# Autodesk Inventor assembly: センサ2セット積み左
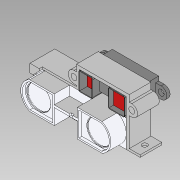
[picture p0: Inventor's stored thumbnail of the model, 180x180]
Saved by Autodesk Inventor 2017 (Build 210142000, 142)
## iProperties
Part Number: センサ2セット積み左
Material: 一般
Document SubType Name: Assembly
Designer: HISAAKI
Author: HISAAKI
## Documents named in this file (4)
- C:\Users\HISAAKI\Documents\LYNCS\CanSat\2017種子島\cansat-structure\センサ2セット積み左.iam
- C:\Users\HISAAKI\Documents\LYNCS\CanSat\2017種子島\cansat-structure\Sharp_2Y0A710.ipt
- C:\Users\HISAAKI\Documents\LYNCS\CanSat\2017種子島\cansat-structure\SharpDistanceRanger.ipt
- C:\Users\HISAAKI\Documents\LYNCS\CanSat\2017種子島\cansat-structure\センサ冶具.ipt
## Components (3 placed, 3 different names)
1. センサ冶具:1 — メイト:1, メイト:2, メイト:3, メイト:4, メイト:5, フラッシュ:1
2. SharpDistanceRanger:1 — メイト:1, メイト:2, メイト:3
3. Sharp_2Y0A710:1 — メイト:4, メイト:5, フラッシュ:1
## Relationships (6: Mate 5, Flush 1)
- メイト:1 [Mate]: センサ冶具:1 ↔ SharpDistanceRanger:1
- メイト:2 [Mate]: センサ冶具:1 ↔ SharpDistanceRanger:1
- メイト:3 [Mate]: センサ冶具:1 ↔ SharpDistanceRanger:1
- メイト:4 [Mate]: センサ冶具:1 ↔ Sharp_2Y0A710:1
- メイト:5 [Mate]: センサ冶具:1 ↔ Sharp_2Y0A710:1
- フラッシュ:1 [Flush]: センサ冶具:1 ↔ Sharp_2Y0A710:1
